# Autodesk Inventor assembly: Shaftside Frame
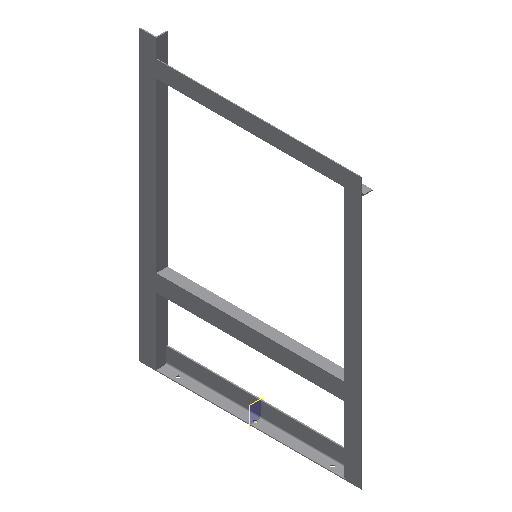
[picture p0: Inventor's stored thumbnail of the model, 512x512]
Saved by Autodesk Inventor 2022 (Build 260148000, 148)
## iProperties
Created: 2007-12-17
Part Number: Shaftside Frame
Document SubType Name: Assembly
Designer: nino.caldarola
Mass: 2990.77 g
Surface Area: 12604.1 cm^2
Volume: 2990.77 cm^3
Density: 1 g/cm^3
_FrameDoc: Frame Assembly
_Version: 25.0.0
Author: nino.caldarola
## Documents named in this file (12)
- D:\Autodesk Inventor 2021 Advanced Assembly Modeling Practice Files\Blower\Shaftside Frame.iam
- D:\Autodesk Inventor 2021 Advanced Assembly Modeling Practice Files\Blower\Shaftside Frame.Skeleton0001.ipt
- D:\Autodesk Inventor 2021 Advanced Assembly Modeling Practice Files\Blower\ANSI L 3 x 2 x 3_16 00000001.ipt
- ANSI L 3 x 2 x 3_16 01.ipt
- D:\Autodesk Inventor 2021 Advanced Assembly Modeling Practice Files\Blower\ANSI L 3 x 2 x 3_16 00000002.ipt
- ANSI L 3 x 2 x 3_16 02.ipt
- D:\Autodesk Inventor 2021 Advanced Assembly Modeling Practice Files\Blower\ANSI L 3 x 2 x 3_16 00000003.ipt
- ANSI L 3 x 2 x 3_16 03.ipt
- D:\Autodesk Inventor 2021 Advanced Assembly Modeling Practice Files\Blower\ANSI L 3 x 2 x 3_16 00000004.ipt
- ANSI L 3 x 2 x 3_16 04.ipt
- D:\Autodesk Inventor 2021 Advanced Assembly Modeling Practice Files\Blower\ANSI L 3 x 2 x 3_16 00000005.ipt
- ANSI L 3 x 2 x 3_16 05.ipt
## Components (6 placed, 6 different names)
1. Frame Reference Model
2. ANSI L 3 x 2 x 3_16 01:1
3. ANSI L 3 x 2 x 3_16 02:1
4. ANSI L 3 x 2 x 3_16 03:1
5. ANSI L 3 x 2 x 3_16 04:1
6. ANSI L 3 x 2 x 3_16 05:1 — Mate:1, Angle:1
## Relationships (2: Mate 1, Angle 1)
- Mate:1: ANSI L 3 x 2 x 3_16 05:1
- Angle:1 (0 deg): ANSI L 3 x 2 x 3_16 05:1
